# Autodesk Inventor assembly: TPU Based Assembly
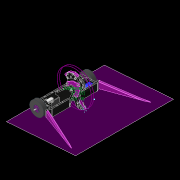
[picture p0: Inventor's stored thumbnail of the model, 180x180]
Saved by Autodesk Inventor 2022 (Build 260153000, 153)
## iProperties
Created: 2022-02-23
Part Number: TPU Based Assembly
Document SubType Name: Assembly
Designer: tandu
Mass: 410.478 g
Surface Area: 1436.98 cm^2
Volume: 270.669 cm^3
Density: 1.51653 g/cm^3
Author: tandu
## Documents named in this file (16)
- C:\Users\tandu\Documents\GrabCAD\Insomnia 2020\Versions\8 Longg forks 8 5 22\TPU Based Assembly 8.iam
- C:\Users\tandu\Documents\GrabCAD\Insomnia 2020\Versions\8 Longg forks 8 5 22\BatteryMockup.ipt
- C:\Users\tandu\Documents\GrabCAD\Insomnia 2020\Versions\8 Longg forks 8 5 22\CorrectSizeWheelsIThink.ipt
- C:\Users\tandu\Documents\GrabCAD\Insomnia 2020\Versions\8 Longg forks 8 5 22\EMax RS2205 v1.ipt
- C:\Users\tandu\Documents\GrabCAD\Insomnia 2020\Versions\8 Longg forks 8 5 22\FingerTech_Silver_Spark_223350.ipt
- C:\Users\tandu\Documents\GrabCAD\Insomnia 2020\Versions\8 Longg forks 8 5 22\TPU 22 Chassis.ipt
- C:\Users\tandu\Documents\GrabCAD\Insomnia 2020\Versions\8 Longg forks 8 5 22\UHMWMotorUpright.ipt
- C:\Users\tandu\Documents\GrabCAD\Insomnia 2020\Versions\8 Longg forks 8 5 22\UHMWBearingUpright.ipt
- C:\Users\tandu\Documents\GrabCAD\Insomnia 2020\Versions\8 Longg forks 8 5 22\Weapon\Aluminimumanfmonfo Jank Weapon Fix.iam
- C:\Users\tandu\Documents\GrabCAD\Insomnia 2020\Versions\8 Longg forks 8 5 22\WedgeUHMWPiece.ipt
- C:\Users\tandu\Documents\GrabCAD\Insomnia 2020\Versions\8 Longg forks 8 5 22\57155K571_Flanged Ball Bearing.ipt
- C:\Users\tandu\Documents\GrabCAD\Insomnia 2020\Versions\8 Longg forks 8 5 22\2207 5 fixed motor.ipt
- C:\Users\tandu\Documents\GrabCAD\Insomnia 2020\Versions\8 Longg forks 8 5 22\WeaponSpacer.ipt
- C:\Users\tandu\Documents\GrabCAD\Insomnia 2020\Versions\8 Longg forks 8 5 22\WedgeUHMWPiece_MIR.ipt
- C:\Users\tandu\Documents\GrabCAD\Insomnia 2020\Versions\8 Longg forks 8 5 22\Derived Lid v8.ipt
- C:\Users\tandu\Documents\GrabCAD\Insomnia 2020\Versions\8 Longg forks 8 5 22\90417A126_Phillips Rounded Head Thread-Forming Screws.ipt
## Components (18 placed, 15 different names)
1. BatteryMockup:1 — Mate:1, Mate:6, Mate:7
2. CorrectSizeWheelsIThink:1 — Insert:2
3. FingerTech_Silver_Spark_223350:1 — Insert:9, Mate:4
4. TPU 22 Chassis:1 — Mate:1, Insert:1, Insert:2, Insert:9, Mate:4, Insert:10, Mate:5, Insert:11, Insert:12, Insert:13, Insert:14, Insert:18, Insert:19, Insert:20, Insert:21, Mate:6, Mate:7, Insert:26, Insert:27
5. FingerTech_Silver_Spark_223350:2 — Insert:10, Mate:5
6. CorrectSizeWheelsIThink:2 — Insert:1, Tangent:1
7. UHMWMotorUpright:1 — Insert:11, Insert:12, Insert:15, Insert:16, Insert:23, Insert:24, Symmetry:1, Insert:28
8. UHMWBearingUpright:1 — Insert:13, Insert:14, Insert:22, Flush:2, Symmetry:1
9. EMax RS2205 v1:1 — Insert:15, Insert:16
10. Aluminimumanfmonfo Jank Weapon Fix:1 [sub-assembly] — Insert:25, Flush:1
11. WedgeUHMWPiece:1 — Insert:20, Insert:21
12. WedgeUHMWPiece:2 — Insert:18, Insert:19, Mate:8
13. 57155K571_Flanged Ball Bearing:1 — Insert:22
14. 2207 5 fixed motor:1 — Insert:23, Insert:24, Insert:25
15. WeaponSpacer:1 — Flush:1, Flush:2
16. WedgePiece_MIR:1 — Mate:9
17. Derived Lid v8:1 — Insert:26, Insert:27
18. 90417A126_Phillips Rounded Head Thread-Forming Screws:1 — Insert:28
## Relationships (33: Insert 21, Mate 8, Flush 2, Symmetry 1, Tangent 1)
- Mate:1: BatteryMockup:1 ↔ TPU 22 Chassis:1
- Insert:1: TPU 22 Chassis:1 ↔ CorrectSizeWheelsIThink:2
- Insert:2: CorrectSizeWheelsIThink:1 ↔ TPU 22 Chassis:1
- Insert:9: FingerTech_Silver_Spark_223350:1 ↔ TPU 22 Chassis:1
- Mate:4: FingerTech_Silver_Spark_223350:1 ↔ TPU 22 Chassis:1
- Insert:10: TPU 22 Chassis:1 ↔ FingerTech_Silver_Spark_223350:2
- Mate:5: TPU 22 Chassis:1 ↔ FingerTech_Silver_Spark_223350:2
- Insert:11: TPU 22 Chassis:1 ↔ UHMWMotorUpright:1
- Insert:12: TPU 22 Chassis:1 ↔ UHMWMotorUpright:1
- Insert:13: TPU 22 Chassis:1 ↔ UHMWBearingUpright:1
- Insert:14: TPU 22 Chassis:1 ↔ UHMWBearingUpright:1
- Insert:15: UHMWMotorUpright:1 ↔ EMax RS2205 v1:1
- Insert:16: UHMWMotorUpright:1 ↔ EMax RS2205 v1:1
- Insert:18: TPU 22 Chassis:1 ↔ WedgeUHMWPiece:2
- Insert:19: TPU 22 Chassis:1 ↔ WedgeUHMWPiece:2
- Insert:20: TPU 22 Chassis:1 ↔ WedgeUHMWPiece:1
- Insert:21: TPU 22 Chassis:1 ↔ WedgeUHMWPiece:1
- Insert:22: UHMWBearingUpright:1 ↔ 57155K571_Flanged Ball Bearing:1
- Insert:23: UHMWMotorUpright:1 ↔ 2207 5 fixed motor:1
- Insert:24: UHMWMotorUpright:1 ↔ 2207 5 fixed motor:1
- Insert:25: Aluminimumanfmonfo Jank Weapon Fix:1 ↔ 2207 5 fixed motor:1
- Flush:1: Aluminimumanfmonfo Jank Weapon Fix:1 ↔ WeaponSpacer:1
- Flush:2: UHMWBearingUpright:1 ↔ WeaponSpacer:1
- Mate:6: BatteryMockup:1 ↔ TPU 22 Chassis:1
- Mate:7: BatteryMockup:1 ↔ TPU 22 Chassis:1
- Symmetry:1: UHMWMotorUpright:1 ↔ UHMWBearingUpright:1
- Mate:8: WedgeUHMWPiece:2
- Mate:9: WedgePiece_MIR:1
- Mate:10
- Tangent:1: CorrectSizeWheelsIThink:2
- Insert:26: TPU 22 Chassis:1 ↔ Derived Lid v8:1
- Insert:27: TPU 22 Chassis:1 ↔ Derived Lid v8:1
- Insert:28: UHMWMotorUpright:1 ↔ 90417A126_Phillips Rounded Head Thread-Forming Screws:1
